# Autodesk Inventor assembly: Baugruppe Ampel
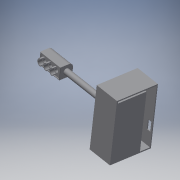
[picture p0: Inventor's stored thumbnail of the model, 180x180]
Saved by Autodesk Inventor 2019.5 (Build 235369000, 369)
## iProperties
Created: 2021-09-30
Part Number: Baugruppe Ampel
Material: Generisch
Document SubType Name: Assembly
Designer: mritt
Author: mritt
## Documents named in this file (3)
- D:\Studium\Universität Stuttgart\Sonstige Tätigkeiten\Tätigkeit_studentische_Hilfskraft_Informatik\Hiwi-Projekt\CAD-Dateien\Arena\Arena Komplettset\Baugruppe Ampel.iam
- D:\Studium\Universität Stuttgart\Sonstige Tätigkeiten\Tätigkeit_studentische_Hilfskraft_Informatik\Hiwi-Projekt\CAD-Dateien\Arena\Arena Komplettset\Battery-Pack-Ampel.ipt
- D:\Studium\Universität Stuttgart\Sonstige Tätigkeiten\Tätigkeit_studentische_Hilfskraft_Informatik\Hiwi-Projekt\CAD-Dateien\Arena\Arena Komplettset\Ampel.ipt
## Components (2 placed, 2 different names)
1. Battery-Pack-Ampel:1 — Fluchtend:1, Passend:1, Passend:2
2. Ampel:1 — Fluchtend:1, Passend:1, Passend:2
## Relationships (3: Mate 2, Flush 1)
- Fluchtend:1 [Flush]: Battery-Pack-Ampel:1 ↔ Ampel:1
- Passend:1 [Mate]: Battery-Pack-Ampel:1 ↔ Ampel:1
- Passend:2 [Mate]: Battery-Pack-Ampel:1 ↔ Ampel:1
